# Autodesk Inventor assembly: wheel_axle
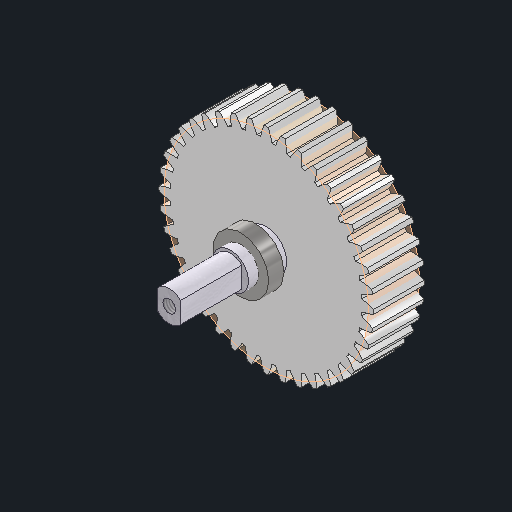
[picture p0: Inventor's stored thumbnail of the model, 512x512]
Saved by Autodesk Inventor 2023 (Build 270158000, 158)
## iProperties
Created: 2024-04-09
Part Number: wheel_axle
Document SubType Name: Assembly
Designer: szymo
Mass: 22 g
Surface Area: 63.6068 cm^2
Volume: 13.7138 cm^3
Density: 1.60422 g/cm^3
TOTAL MASS: 0.0
Author: szymo
## Documents named in this file (6)
- D:\roboilo\robots\codename wafel - australia\3d_parts\rev4\wheel_axle.iam
- D:\roboilo\robots\codename wafel - australia\3d_parts\rev4\MegaSumo kola zebate 38.ipt
- D:\roboilo\robots\codename wafel - australia\3d_parts\rev4\wal_kola.ipt
- D:\roboilo\robots\codename wafel - australia\3d_parts\rev4\small_bearing.ipt
- D:\roboilo\robots\codename wafel - australia\3d_parts\rev4\big_bearing.ipt
- D:\roboilo\robots\codename wafel - australia\3d_parts\rev4\Design Accelerator\big_gear3.iam
## Components (5 placed, 5 different names)
1. wal_kola:1 — Rotational:1, Mate:3, Mate:4, Mate:5, Mate:6, Angle:1
2. MegaSumo kola zebate 38:1 — Rotational:1, Flush:1, Mate:7
3. small_bearing:1 — Mate:3, Mate:4
4. big_bearing:1 — Mate:5, Mate:6
5. big_gear:1 [sub-assembly] — Flush:1, Mate:7, Angle:1
## Relationships (8: Mate 5, RevoluteJoint 1, Flush 1, Angle 1)
- Rotational:1 [RevoluteJoint]: wal_kola:1 ↔ MegaSumo kola zebate 38:1
- Mate:3: wal_kola:1 ↔ small_bearing:1
- Mate:4: wal_kola:1 ↔ small_bearing:1
- Mate:5: wal_kola:1 ↔ big_bearing:1
- Mate:6: wal_kola:1 ↔ big_bearing:1
- Flush:1: MegaSumo kola zebate 38:1 ↔ big_gear:1
- Mate:7: MegaSumo kola zebate 38:1 ↔ big_gear:1
- Angle:1 (0 deg): wal_kola:1 ↔ big_gear:1
